# Autodesk Inventor assembly: gripper_testing
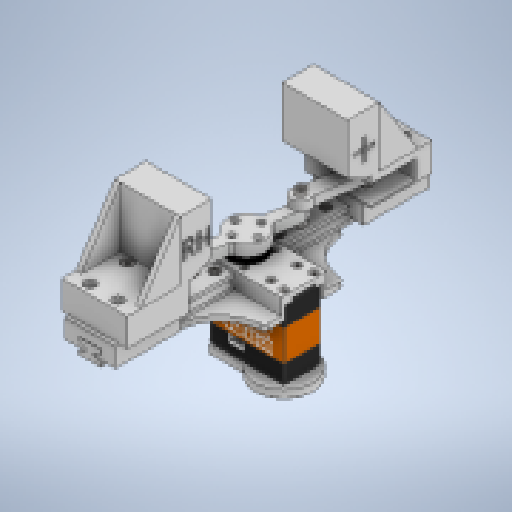
[picture p0: Inventor's stored thumbnail of the model, 512x512]
Saved by Autodesk Inventor 2024 (Build 280153000, 153)
## iProperties
Created: 2023-10-13
Part Number: gripper_testing
Document SubType Name: Assembly
Designer: 박동준
Author: 박동준
## Documents named in this file (16)
- C:\Users\박동준\OneDrive - 연세대학교 (Yonsei University)\바탕 화면\박동준\대학생할\로봇\Humanoid\7축 매니퓰레이터\하드웨어\rh_plus_7_axis_robot_arm_hardware\Assembly\3_Gripper.iam
- C:\Users\박동준\OneDrive - 연세대학교 (Yonsei University)\바탕 화면\박동준\대학생할\로봇\Humanoid\7축 매니퓰레이터\하드웨어\rh_plus_7_axis_robot_arm_hardware\Part\Frame\gripper\gripper.ipt
- C:\Users\박동준\OneDrive - 연세대학교 (Yonsei University)\바탕 화면\박동준\대학생할\로봇\Humanoid\7축 매니퓰레이터\하드웨어\rh_plus_7_axis_robot_arm_hardware\Part\Frame\gripper\gripper_base_frame.ipt
- C:\Users\박동준\OneDrive - 연세대학교 (Yonsei University)\바탕 화면\박동준\대학생할\로봇\Humanoid\7축 매니퓰레이터\하드웨어\rh_plus_7_axis_robot_arm_hardware\Part\Frame\axis_7_top_frame.ipt
- C:\Users\박동준\OneDrive - 연세대학교 (Yonsei University)\바탕 화면\박동준\대학생할\로봇\Humanoid\7축 매니퓰레이터\하드웨어\rh_plus_7_axis_robot_arm_hardware\Part\Frame\gripper\gripper_hand_connector.ipt
- C:\Users\박동준\OneDrive - 연세대학교 (Yonsei University)\바탕 화면\박동준\대학생할\로봇\Humanoid\7축 매니퓰레이터\하드웨어\rh_plus_7_axis_robot_arm_hardware\Part\Other Parts\lm_guide_cart.ipt
- C:\Users\박동준\OneDrive - 연세대학교 (Yonsei University)\바탕 화면\박동준\대학생할\로봇\Humanoid\7축 매니퓰레이터\하드웨어\rh_plus_7_axis_robot_arm_hardware\Part\Other Parts\lm_guide_rail.ipt
- C:\Users\박동준\OneDrive - 연세대학교 (Yonsei University)\바탕 화면\박동준\대학생할\로봇\Humanoid\7축 매니퓰레이터\하드웨어\rh_plus_7_axis_robot_arm_hardware\Part\HTD-45H, Horn\HTD-45H\HTD-45H.iam
- C:\Users\박동준\OneDrive - 연세대학교 (Yonsei University)\바탕 화면\박동준\대학생할\로봇\Humanoid\7축 매니퓰레이터\하드웨어\rh_plus_7_axis_robot_arm_hardware\Part\HTD-45H, Horn\Horn\Top Horn.ipt
- C:\Users\박동준\OneDrive - 연세대학교 (Yonsei University)\바탕 화면\박동준\대학생할\로봇\Humanoid\7축 매니퓰레이터\하드웨어\rh_plus_7_axis_robot_arm_hardware\Part\Bolt, Bearing, Nut, Washer\M3x8.ipt
- C:\Users\박동준\OneDrive - 연세대학교 (Yonsei University)\바탕 화면\박동준\대학생할\로봇\Humanoid\7축 매니퓰레이터\하드웨어\rh_plus_7_axis_robot_arm_hardware\Part\Frame\axis_7_bottom_frame.ipt
- C:\Users\박동준\OneDrive - 연세대학교 (Yonsei University)\바탕 화면\박동준\대학생할\로봇\Humanoid\7축 매니퓰레이터\하드웨어\rh_plus_7_axis_robot_arm_hardware\Part\Bolt, Bearing, Nut, Washer\2030 Teflon Sheet.ipt
- C:\Users\박동준\OneDrive - 연세대학교 (Yonsei University)\바탕 화면\박동준\대학생할\로봇\Humanoid\7축 매니퓰레이터\하드웨어\rh_plus_7_axis_robot_arm_hardware\Part\Bolt, Bearing, Nut, Washer\M2x6 Round Bolt.ipt
- C:\Users\박동준\OneDrive - 연세대학교 (Yonsei University)\바탕 화면\박동준\대학생할\로봇\Humanoid\7축 매니퓰레이터\하드웨어\rh_plus_7_axis_robot_arm_hardware\Part\Bolt, Bearing, Nut, Washer\M3x15.ipt
- C:\Users\박동준\OneDrive - 연세대학교 (Yonsei University)\바탕 화면\박동준\대학생할\로봇\Humanoid\7축 매니퓰레이터\하드웨어\rh_plus_7_axis_robot_arm_hardware\Part\Bolt, Bearing, Nut, Washer\M3x10.ipt
- C:\Users\박동준\OneDrive - 연세대학교 (Yonsei University)\바탕 화면\박동준\대학생할\로봇\Humanoid\7축 매니퓰레이터\하드웨어\rh_plus_7_axis_robot_arm_hardware\Part\Bolt, Bearing, Nut, Washer\M3 Nylon Nut.ipt
## Components (50 placed, 15 different names)
1. M3x10:2 — Mate:88, Mate:95, Mate:97
2. M3x10:1 — Rigid:22
3. M3x8:1 — Rotational:13
4. M3x8:2 — Rotational:14
5. M3x8:3 — Rotational:16
6. M3x8:4 — Rotational:15
7. M3x8:7 — Mate:65, Mate:66
8. M3x8:8 — Mate:61, Mate:62
9. M3x8:9 — Mate:63, Mate:64
10. M3x8:10 — Mate:87, Mate:90, Mate:92
11. M3x8:11 — Mate:89, Mate:94, Mate:98
12. M3x8:12 — Mate:86, Mate:91, Mate:93
13. M3x15:1 — Mate:77, Mate:80
14. M3x15:2 — Mate:78, Mate:79
15. M2x6 Round Bolt:1 — Rigid:2
16. M2x6 Round Bolt:2 — Rigid:4
17. M2x6 Round Bolt:3 — Rigid:6
18. M2x6 Round Bolt:4 — Rigid:11
19. M2x6 Round Bolt:5 — Rigid:3
20. M2x6 Round Bolt:6 — Rigid:7
21. M2x6 Round Bolt:7 — Rigid:8
22. M2x6 Round Bolt:8 — Rigid:5
23. M2x6 Round Bolt:9 — Rigid:10
24. M2x6 Round Bolt:10 — Rigid:9
25. M2x6 Round Bolt:11 — Rotational:24
26. M2x6 Round Bolt:12 — Rotational:25
27. M2x6 Round Bolt:13 — Rigid:28
28. M2x6 Round Bolt:14 — Rotational:22
29. M2x6 Round Bolt:15 — Rotational:23
30. M2x6 Round Bolt:16 — Rigid:30
31. M2x6 Round Bolt:17 — Rigid:29
32. M2x6 Round Bolt:18 — Rigid:31
33. M3 Nylon Nut:1 — Rigid:24
34. M3 Nylon Nut:2 — Rigid:25
35. M3 Nylon Nut:3 — Rigid:26
36. M3 Nylon Nut:4 — Rigid:27
37. gripper_base_frame:2 — Rigid:21, Mate:81, Mate:82, Rigid:25, Rigid:26, Mate:85
38. 2030 Teflon Sheet:1 — Rigid:12
39. axis_7_top_frame:1 — Mate:11, Angle:1, Mate:12, Mate:13, Mate:14, Mate:15, Mate:16, Mate:17, Mate:99, Rigid:28, Rigid:29, Rigid:31, Rigid:30, Rotational:22, Rotational:23, Rotational:24, Rotational:25
40. axis_7_bottom_frame:1 — Rigid:1, Rigid:2, Rigid:3, Rigid:4, Rigid:5, Rigid:6, Rigid:7, Rigid:8, Rigid:9, Rigid:10, Rigid:11, Rigid:12
41. HTD-45H:1 [sub-assembly] — Mate:11, Angle:1, Mate:49, Flush:2, Flush:3, Rigid:1, Rotational:21
42. Top Horn:1 — Rotational:21, Rigid:21, Mate:99
43. gripper:1 — Angle:4, Mate:44, Mate:50, Mate:51, Mate:61, Mate:62, Mate:63, Mate:64, Mate:65, Mate:66, Rigid:22
44. gripper:2 — Angle:5, Mate:90, Mate:91, Mate:92, Mate:93, Mate:94, Mate:95, Mate:96, Mate:98
45. gripper_hand_connector:1 — Mate:77, Mate:80, Mate:81, Rigid:24, Mate:85, Mate:97
46. gripper_hand_connector:2 — Mate:51, Mate:78, Mate:79, Mate:82, Rigid:27
47. lm_guide_cart:1 — Mate:18, Angle:2, Mate:19, Mate:86, Mate:87, Mate:88, Mate:89, Angle:5, Mate:96
48. lm_guide_cart:2 — Mate:20, Angle:3, Mate:21, Angle:4, Mate:44, Mate:50
49. lm_guide_rail:1 — Mate:12, Mate:13, Mate:14, Mate:18, Angle:2, Mate:19, Rotational:13, Rotational:14
50. lm_guide_rail:2 — Mate:15, Mate:16, Mate:17, Mate:20, Angle:3, Mate:21, Rotational:15, Rotational:16
## Relationships (80: Mate 42, WeldJoint 22, RevoluteJoint 9, Angle 5, Flush 2)
- Mate:11: axis_7_top_frame:1 ↔ HTD-45H:1
- Angle:1 (0 deg): axis_7_top_frame:1 ↔ HTD-45H:1
- Mate:12: axis_7_top_frame:1 ↔ lm_guide_rail:1
- Mate:13: axis_7_top_frame:1 ↔ lm_guide_rail:1
- Mate:14: axis_7_top_frame:1 ↔ lm_guide_rail:1
- Mate:15: axis_7_top_frame:1 ↔ lm_guide_rail:2
- Mate:16: axis_7_top_frame:1 ↔ lm_guide_rail:2
- Mate:17: axis_7_top_frame:1 ↔ lm_guide_rail:2
- Mate:18: lm_guide_cart:1 ↔ lm_guide_rail:1
- Angle:2 (0 deg): lm_guide_cart:1 ↔ lm_guide_rail:1
- Mate:19: lm_guide_cart:1 ↔ lm_guide_rail:1
- Mate:20: lm_guide_cart:2 ↔ lm_guide_rail:2
- Angle:3 (0 deg): lm_guide_cart:2 ↔ lm_guide_rail:2
- Mate:21: lm_guide_cart:2 ↔ lm_guide_rail:2
- Angle:4 (0 deg): gripper:1 ↔ lm_guide_cart:2
- Rotational:13 [RevoluteJoint]: M3x8:1 ↔ lm_guide_rail:1
- Rotational:14 [RevoluteJoint]: M3x8:2 ↔ lm_guide_rail:1
- Rotational:15 [RevoluteJoint]: M3x8:4 ↔ lm_guide_rail:2
- Mate:44: gripper:1 ↔ lm_guide_cart:2
- Rotational:16 [RevoluteJoint]: M3x8:3 ↔ lm_guide_rail:2
- Mate:49: HTD-45H:1
- Flush:2: HTD-45H:1
- Flush:3: HTD-45H:1
- Rigid:1 [WeldJoint]: axis_7_bottom_frame:1 ↔ HTD-45H:1
- Rigid:2 [WeldJoint]: M2x6 Round Bolt:1 ↔ axis_7_bottom_frame:1
- Rigid:3 [WeldJoint]: M2x6 Round Bolt:5 ↔ axis_7_bottom_frame:1
- Rigid:4 [WeldJoint]: M2x6 Round Bolt:2 ↔ axis_7_bottom_frame:1
- Rigid:5 [WeldJoint]: M2x6 Round Bolt:8 ↔ axis_7_bottom_frame:1
- Rigid:6 [WeldJoint]: M2x6 Round Bolt:3 ↔ axis_7_bottom_frame:1
- Rigid:7 [WeldJoint]: M2x6 Round Bolt:6 ↔ axis_7_bottom_frame:1
- Rigid:8 [WeldJoint]: M2x6 Round Bolt:7 ↔ axis_7_bottom_frame:1
- Rigid:9 [WeldJoint]: M2x6 Round Bolt:10 ↔ axis_7_bottom_frame:1
- Rigid:10 [WeldJoint]: M2x6 Round Bolt:9 ↔ axis_7_bottom_frame:1
- Rigid:11 [WeldJoint]: M2x6 Round Bolt:4 ↔ axis_7_bottom_frame:1
- Rigid:12 [WeldJoint]: 2030 Teflon Sheet:1 ↔ axis_7_bottom_frame:1
- Mate:50: gripper:1 ↔ lm_guide_cart:2
- Mate:51: gripper:1 ↔ gripper_hand_connector:2
- Mate:61: M3x8:8 ↔ gripper:1
- Mate:62: M3x8:8 ↔ gripper:1
- Mate:63: M3x8:9 ↔ gripper:1
- Mate:64: M3x8:9 ↔ gripper:1
- Mate:65: M3x8:7 ↔ gripper:1
- Mate:66: M3x8:7 ↔ gripper:1
- Mate:77: M3x15:1 ↔ gripper_hand_connector:1
- Mate:78: M3x15:2 ↔ gripper_hand_connector:2
- Mate:79: M3x15:2 ↔ gripper_hand_connector:2
- Mate:80: M3x15:1 ↔ gripper_hand_connector:1
- Rotational:21 [RevoluteJoint]: HTD-45H:1 ↔ Top Horn:1
- Rigid:21 [WeldJoint]: gripper_base_frame:2 ↔ Top Horn:1
- Mate:81: gripper_base_frame:2 ↔ gripper_hand_connector:1
- Mate:82: gripper_base_frame:2 ↔ gripper_hand_connector:2
- Rigid:22 [WeldJoint]: M3x10:1 ↔ gripper:1
- Rigid:24 [WeldJoint]: M3 Nylon Nut:1 ↔ gripper_hand_connector:1
- Rigid:25 [WeldJoint]: M3 Nylon Nut:2 ↔ gripper_base_frame:2
- Rigid:26 [WeldJoint]: M3 Nylon Nut:3 ↔ gripper_base_frame:2
- Rigid:27 [WeldJoint]: M3 Nylon Nut:4 ↔ gripper_hand_connector:2
- Mate:85: gripper_base_frame:2 ↔ gripper_hand_connector:1
- Mate:86: M3x8:12 ↔ lm_guide_cart:1
- Mate:87: M3x8:10 ↔ lm_guide_cart:1
- Mate:88: M3x10:2 ↔ lm_guide_cart:1
- Mate:89: M3x8:11 ↔ lm_guide_cart:1
- Angle:5 (0 deg): gripper:2 ↔ lm_guide_cart:1
- Mate:90: M3x8:10 ↔ gripper:2
- Mate:91: M3x8:12 ↔ gripper:2
- Mate:92: M3x8:10 ↔ gripper:2
- Mate:93: M3x8:12 ↔ gripper:2
- Mate:94: M3x8:11 ↔ gripper:2
- Mate:95: M3x10:2 ↔ gripper:2
- Mate:96: gripper:2 ↔ lm_guide_cart:1
- Mate:97: M3x10:2 ↔ gripper_hand_connector:1
- Mate:98: M3x8:11 ↔ gripper:2
- Mate:99: axis_7_top_frame:1 ↔ Top Horn:1
- Rigid:28 [WeldJoint]: M2x6 Round Bolt:13 ↔ axis_7_top_frame:1
- Rigid:29 [WeldJoint]: M2x6 Round Bolt:17 ↔ axis_7_top_frame:1
- Rigid:31 [WeldJoint]: M2x6 Round Bolt:18 ↔ axis_7_top_frame:1
- Rigid:30 [WeldJoint]: M2x6 Round Bolt:16 ↔ axis_7_top_frame:1
- Rotational:22 [RevoluteJoint]: M2x6 Round Bolt:14 ↔ axis_7_top_frame:1
- Rotational:23 [RevoluteJoint]: M2x6 Round Bolt:15 ↔ axis_7_top_frame:1
- Rotational:24 [RevoluteJoint]: M2x6 Round Bolt:11 ↔ axis_7_top_frame:1
- Rotational:25 [RevoluteJoint]: M2x6 Round Bolt:12 ↔ axis_7_top_frame:1
